# Autodesk Inventor assembly: CFflange Assly 01
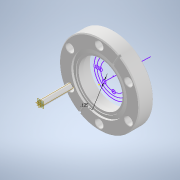
[picture p0: Inventor's stored thumbnail of the model, 180x180]
Saved by Autodesk Inventor 2020 (Build 240168000, 168)
## iProperties
Created: 2019-05-09
Part Number: CFflange Assly 01
Document SubType Name: Assembly
Designer: isadmin
Author: isadmin
## Documents named in this file (3)
- C:\Users\isadmin\Documents\Inventor\IS_01\CFflange Assly 01.iam
- C:\Users\isadmin\Documents\Inventor\IS_01\FlangeCF275 Bored_1112112 REV 1 .ipt
- C:\Users\isadmin\Documents\Inventor\IS_01\support_rod_ebeam_heater_v0.ipt
## Components (2 placed, 2 different names)
1. FlangeCF275 Bored_1112112 REV 1 :1 — Mate:1, Mate:2
2. support_rod_ebeam_heater_v0:1 — Mate:1, Mate:2
## Relationships (2: Mate 2)
- Mate:1: FlangeCF275 Bored_1112112 REV 1 :1 ↔ support_rod_ebeam_heater_v0:1
- Mate:2: FlangeCF275 Bored_1112112 REV 1 :1 ↔ support_rod_ebeam_heater_v0:1
